# Autodesk Inventor assembly: Cơ cấu gạt cốc
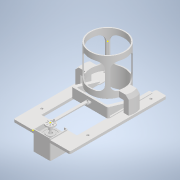
[picture p0: Inventor's stored thumbnail of the model, 180x180]
Saved by Autodesk Inventor 2020 (Build 240168000, 168)
## iProperties
Created: 2022-11-23
Part Number: Cơ cấu gạt cốc
Document SubType Name: Assembly
Designer: ADMIN
Author: ADMIN
## Documents named in this file (8)
- D:\Do-an-tot-nghiep\Inventor\Cơ cấu gạt cốc.iam
- D:\Do-an-tot-nghiep\Inventor\Hộp đựng động cơ.ipt
- D:\Do-an-tot-nghiep\Inventor\Khay đựng cốc.ipt
- D:\Do-an-tot-nghiep\Inventor\Khay gạt cốc.ipt
- D:\Do-an-tot-nghiep\Inventor\tay quay.ipt
- C:\Users\ADMIN\Documents\Inventor\Content Center Files\R2020\en-US\ISO 2338(2)\ISO 2338 - 4 h8 x 8.ipt
- D:\Do-an-tot-nghiep\Inventor\step\Assembly1.iam
- D:\Do-an-tot-nghiep\Inventor\trục quay.ipt
## Components (8 placed, 7 different names)
1. Hộp đựng động cơ:1 — Mate:1, Mate:6, Mate:7, Mate:8, Mate:13, Mate:14, Mate:15
2. Khay đựng cốc:1 — Mate:1, Mate:14, Mate:15
3. Khay gạt cốc:1 — Mate:3, Mate:4, Mate:13
4. tay quay:1 — Mate:3, Mate:4, Mate:5, Flush:1, Mate:10, Mate:11, Mate:12, Flush:3
5. ISO 2338 4 h8 x 8:1 — Mate:5, Flush:1
6. Assembly1:1 [sub-assembly] — Mate:6, Mate:7, Mate:8, Mate:9
7. trục quay:1 — Mate:9, Mate:10, Mate:11
8. ISO 2338 4 h8 x 8:2 — Mate:12, Flush:3
## Relationships (16: Mate 14, Flush 2)
- Mate:1: Hộp đựng động cơ:1 ↔ Khay đựng cốc:1
- Mate:3: Khay gạt cốc:1 ↔ tay quay:1
- Mate:4: Khay gạt cốc:1 ↔ tay quay:1
- Mate:5: tay quay:1 ↔ ISO 2338 4 h8 x 8:1
- Mate:6: Hộp đựng động cơ:1 ↔ Assembly1:1
- Mate:7: Hộp đựng động cơ:1 ↔ Assembly1:1
- Flush:1: tay quay:1 ↔ ISO 2338 4 h8 x 8:1
- Mate:8: Hộp đựng động cơ:1 ↔ Assembly1:1
- Mate:9: Assembly1:1 ↔ trục quay:1
- Mate:10: tay quay:1 ↔ trục quay:1
- Mate:11: tay quay:1 ↔ trục quay:1
- Mate:12: tay quay:1 ↔ ISO 2338 4 h8 x 8:2
- Flush:3: tay quay:1 ↔ ISO 2338 4 h8 x 8:2
- Mate:13: Hộp đựng động cơ:1 ↔ Khay gạt cốc:1
- Mate:14: Hộp đựng động cơ:1 ↔ Khay đựng cốc:1
- Mate:15: Hộp đựng động cơ:1 ↔ Khay đựng cốc:1
